# Autodesk Inventor assembly: UmlenkrolleHalterEinfachAngle
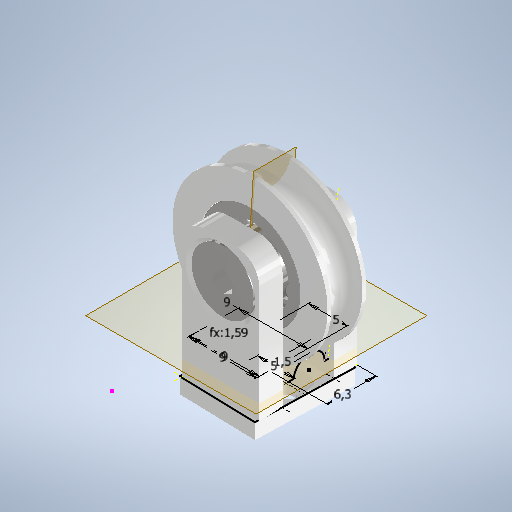
[picture p0: Inventor's stored thumbnail of the model, 512x512]
Saved by Autodesk Inventor 2025 (Build 290162010, 162A)
## iProperties
Created: 2024-11-19
Part Number: UmlenkrolleHalterEinfachAngle
Document SubType Name: Assembly
Designer: Admin
Mass: 6.79388 g
Surface Area: 35.0539 cm^2
Volume: 2.35136 cm^3
Density: 2.88934 g/cm^3
Author: Admin
## Documents named in this file (5)
- C:\Users\Admin\GIT\HDVKBM\CAD\Krandemonstrator\UmlenkrolleHalterEinfachAngle.iam
- C:\Users\Admin\GIT\HDVKBM\CAD\Krandemonstrator\HalterUmlenkrolleOVL.ipt
- C:\Users\Admin\GIT\HDVKBM\CAD\Krandemonstrator\Umlenkrolle.iam
- C:\Users\Admin\Documents\Inventor\Content Center Files\R2025\de-DE\AS 1237 (2.1)\AS 1237 - 4.ipt
- C:\Users\Admin\Documents\Inventor\Content Center Files\R2025\de-DE\DIN 7991(2)\DIN 7991 - M4x12.ipt
## Components (5 placed, 4 different names)
1. HalterUmlenkrolleOVL:1 — Starr:1, Drehbar:1, Drehbar:2
2. Umlenkrolle:1 [sub-assembly] — Drehbar:5
3. DIN 7991 M4x12:1 — Starr:1, Drehbar:5
4. AS 1237 (2.1) 4:1 — Drehbar:2
5. AS 1237 (2.1) 4:2 — Drehbar:1
## Relationships (4: RevoluteJoint 3, WeldJoint 1)
- Starr:1 [WeldJoint]: HalterUmlenkrolleOVL:1 ↔ DIN 7991 M4x12:1
- Drehbar:1 [RevoluteJoint]: HalterUmlenkrolleOVL:1 ↔ AS 1237 (2.1) 4:2
- Drehbar:2 [RevoluteJoint]: HalterUmlenkrolleOVL:1 ↔ AS 1237 (2.1) 4:1
- Drehbar:5 [RevoluteJoint] (-3.275 mm): Umlenkrolle:1 ↔ DIN 7991 M4x12:1
